# Autodesk Inventor assembly: Cylinder Assembly
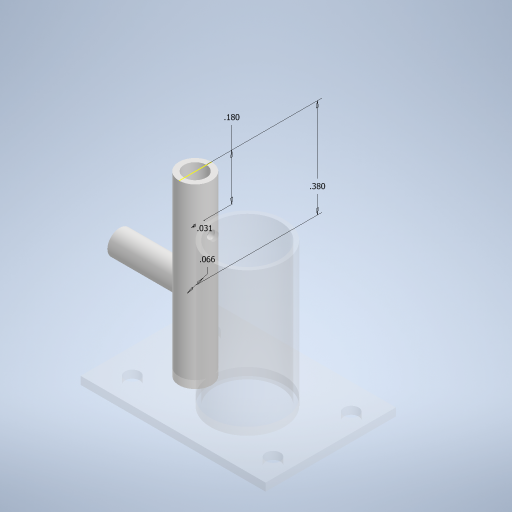
[picture p0: Inventor's stored thumbnail of the model, 512x512]
Saved by Autodesk Inventor 2023 (Build 270158000, 158)
## iProperties
Created: 2023-02-13
Part Number: Cylinder Assembly
Document SubType Name: Assembly
Designer: tommy
Author: tommy
## Documents named in this file (5)
- C:\Users\tommy\Documents\Repositories\Steam-Engine\Les Proper Steam Engine\CAD\Cylinder Assembly.iam
- C:\Users\tommy\Documents\Repositories\Steam-Engine\Les Proper Steam Engine\CAD\Base Top.ipt
- C:\Users\tommy\Documents\Repositories\Steam-Engine\Les Proper Steam Engine\CAD\Inlet Manifold.ipt
- C:\Users\tommy\Documents\Repositories\Steam-Engine\Les Proper Steam Engine\CAD\Valve Tube.ipt
- C:\Users\tommy\Documents\Repositories\Steam-Engine\Les Proper Steam Engine\CAD\Cylinder.ipt
## Components (4 placed, 4 different names)
1. Base Top:1 — Mate:2, Flush:1, Angle:1, Flush:2, Mate:3
2. Inlet Manifold:1 — Mate:1, Angle:1, Mate:4
3. Valve Tube:1 — Mate:1, Mate:2, Flush:1, Mate:4, Mate:5
4. Cylinder:1 — Flush:2, Mate:3, Mate:5
## Relationships (8: Mate 5, Flush 2, Angle 1)
- Mate:1: Inlet Manifold:1 ↔ Valve Tube:1
- Mate:2: Base Top:1 ↔ Valve Tube:1
- Flush:1: Base Top:1 ↔ Valve Tube:1
- Angle:1 (180 deg): Base Top:1 ↔ Inlet Manifold:1
- Flush:2: Base Top:1 ↔ Cylinder:1
- Mate:3: Base Top:1 ↔ Cylinder:1
- Mate:4: Inlet Manifold:1 ↔ Valve Tube:1
- Mate:5: Valve Tube:1 ↔ Cylinder:1
